# Autodesk Inventor assembly: 19197 DSNU-12-200-P-A---(0)
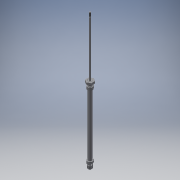
[picture p0: Inventor's stored thumbnail of the model, 180x180]
Saved by Autodesk Inventor 2018 (Build 220112000, 112)
## iProperties
Category: PARTsolutions
Company: FESTO
Created: 2019-05-10
Part Number: 19197 DSNU-12-200-P-A---(0)
Catalog Web Link: www.cadenas.de
Description: DSNU-Round cylinder
Vendor: FESTO
Document SubType Name: Assembly
Designer: psadmin
Manufacturer: FESTO
Mass: 155 g
PSOL_IDENT_0: {ATYP=ASSISTANT},{DATA=script=$CADENAS_DATA/23d-libs/festo/webfesto.vbb/&M_FAMILY=DSNU&M_GROUP=01&M_
PSOL_IDENT_1: PARTNO=19197&IDCODE1=DSNU-12-200-P-A&IDCODE2=&customer_number_cns=&MATES=1&LOD=HI&LOCKERP=0&SINGLEPA
PSOL_IDENT_2: RT=1}
NN: DSNU
NT: Round cylinder
NB: 19197 DSNU-12-200-P-A---(0)
NBSYN: $NB1.---($HUBST.)
LINA: 19197 DSNU-12-200-P-A
OFFICIAL_STANDARD_NUMBERS: ISO 6432
TNR: 19197
TYP: DSNU-12
KDM: 12
HUB: 200
HUBST: 0
DA: P
PE: A
KS: -
A1: 20
A2: 100
A3: 4
A4: 38
AB: 16
AM: 16
B: 16
BB: 3
BE: M16x1,5
BS: 4.5
B1: 30
B2: 0
B3: 0
B4: 0
B5: 18.1
B6: 8
B7: 0
CD: 6
D: 20
D1: 16
D2: 6
D3: 13.3
D4: 5.5
D5: 14.5
D6: 0
D7: 0
EE: M5
EW: 12
F: 23
FF: M4
F1: 0
H: 22
H1: 0
KK: M6
K1: -
K2: 0
KV: 24
KW: 8
KV2: 0
KW2: 0
L: 9
LH: 6
LK: 7.7
L1: 289
L2: 250
L3: 6
L4: 17
L5: 15
L6: 38
L7: 21
L8: 10
L9: 23
L13: 94
ST: 4.5
SW: 5
T: 0
WH: 22
X: 0
XC: 275
CNSMASSEXACT: 0.155
SUPPLIER: FESTO
ARTICLENO: 19197 DSNU-12-200-P-A---(0)
BOMINFO: 19197 DSNU-12-200-P-A
CREATOR: CADENAS GmbH
Title: 19197 DSNU-12-200-P-A
Author: Cadenas PARTsolutions
Comments: Round cylinder
## Documents named in this file (4)
- C:\Users\aal_9\OneDrive\Documentos\Suiza\Courses\Tesis\TestBench\AIS2017\19197 DSNU-12-200-P-A---(0).iam
- C:\Users\aal_9\OneDrive\Documentos\Suiza\Courses\Tesis\TestBench\AIS2017\19197 DSNU-12-200-P---(A----0-ZR).ipt
- C:\Users\aal_9\OneDrive\Documentos\Suiza\Courses\Tesis\TestBench\AIS2017\DIN-439-B - M16x1_5(F).ipt
- C:\Users\aal_9\OneDrive\Documentos\Suiza\Courses\Tesis\TestBench\AIS2017\19197 DSNU-12-200-P---(A---00--0-KS).ipt
## Components (3 placed, 3 different names)
1. 19197 DSNU-12-200-P---(A----0-ZR):1 — NUT_XY@1 <-> 2CYL_XY@2, NUT_Z@1 <-> 2CYL_Z@2, NUT_YZ@1 <-> 2CYL_YZ@2, Cylindrical:1, Mate:3
2. DIN-439-B - M16x1_5(F):1 — NUT_XY@1 <-> 2CYL_XY@2, NUT_Z@1 <-> 2CYL_Z@2, NUT_YZ@1 <-> 2CYL_YZ@2
3. 19197 DSNU-12-200-P---(A---00--0-KS):1 — Cylindrical:1, Mate:3
## Relationships (5: Mate 3, Angle 1, CylindricalJoint 1)
- NUT_XY@1 <-> 2CYL_XY@2 [Mate] (-4 mm): 19197 DSNU-12-200-P---(A----0-ZR):1 ↔ DIN-439-B - M16x1_5(F):1
- NUT_Z@1 <-> 2CYL_Z@2 [Mate]: 19197 DSNU-12-200-P---(A----0-ZR):1 ↔ DIN-439-B - M16x1_5(F):1
- NUT_YZ@1 <-> 2CYL_YZ@2 [Angle] (0 deg): 19197 DSNU-12-200-P---(A----0-ZR):1 ↔ DIN-439-B - M16x1_5(F):1
- Cylindrical:1: 19197 DSNU-12-200-P---(A----0-ZR):1 ↔ 19197 DSNU-12-200-P---(A---00--0-KS):1
- Mate:3 (200 mm): 19197 DSNU-12-200-P---(A----0-ZR):1 ↔ 19197 DSNU-12-200-P---(A---00--0-KS):1
